# Autodesk Inventor assembly: kayboard
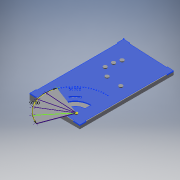
[picture p0: Inventor's stored thumbnail of the model, 180x180]
Saved by Autodesk Inventor 2016 SP2 (Build 200236200, 236)
## iProperties
Created: 2017-09-03
Part Number: kayboard
Document SubType Name: Assembly
Designer: Kartikye
Author: Kartikye
## Documents named in this file (8)
- D:\Documents\cs294\keyboard\kayboard.iam
- D:\Documents\cs294\keyboard\main board.ipt
- D:\Documents\cs294\keyboard\swiweller.ipt
- D:\Documents\cs294\keyboard\side board.ipt
- D:\Documents\cs294\keyboard\bottom.ipt
- D:\Documents\cs294\keyboard\button.iam
- D:\Documents\cs294\keyboard\back.ipt
- D:\Documents\cs294\keyboard\front.ipt
## Components (12 placed, 7 different names)
1. swiweller:1 — Insert:1
2. main board:1 — Insert:1, Mate:1, Flush:1, Mate:2, Mate:3, Flush:2, Mate:4, Insert:2, Insert:3, Insert:4, Insert:5, Insert:6
3. side board:1 — Mate:1, Flush:1, Mate:2
4. side board:2 — Mate:3, Flush:2, Mate:4, Mate:5, Flush:3, Mate:6
5. bottom:1 — Mate:5, Flush:3, Mate:6, Mate:7, Mate:8, Mate:9, Mate:10, Mate:11, Mate:12
6. button:1 [sub-assembly] — Insert:5
7. button:2 [sub-assembly] — Insert:6
8. button:3 [sub-assembly] — Insert:4
9. button:4 [sub-assembly] — Insert:3
10. button:5 [sub-assembly] — Insert:2
11. back:1 — Mate:7, Mate:8, Mate:9
12. front:1 — Mate:10, Mate:11, Mate:12
## Relationships (21: Mate 12, Insert 6, Flush 3)
- Insert:1: swiweller:1 ↔ main board:1
- Mate:1: main board:1 ↔ side board:1
- Flush:1: main board:1 ↔ side board:1
- Mate:2: main board:1 ↔ side board:1
- Mate:3: main board:1 ↔ side board:2
- Flush:2: main board:1 ↔ side board:2
- Mate:4: main board:1 ↔ side board:2
- Mate:5: side board:2 ↔ bottom:1
- Flush:3: side board:2 ↔ bottom:1
- Mate:6: side board:2 ↔ bottom:1
- Insert:2: main board:1 ↔ button:5
- Insert:3: main board:1 ↔ button:4
- Insert:4: main board:1 ↔ button:3
- Insert:5: main board:1 ↔ button:1
- Insert:6: main board:1 ↔ button:2
- Mate:7: bottom:1 ↔ back:1
- Mate:8: bottom:1 ↔ back:1
- Mate:9: bottom:1 ↔ back:1
- Mate:10: bottom:1 ↔ front:1
- Mate:11: bottom:1 ↔ front:1
- Mate:12: bottom:1 ↔ front:1
